# Autodesk Inventor assembly: Tamale - V1p5 - keepouts
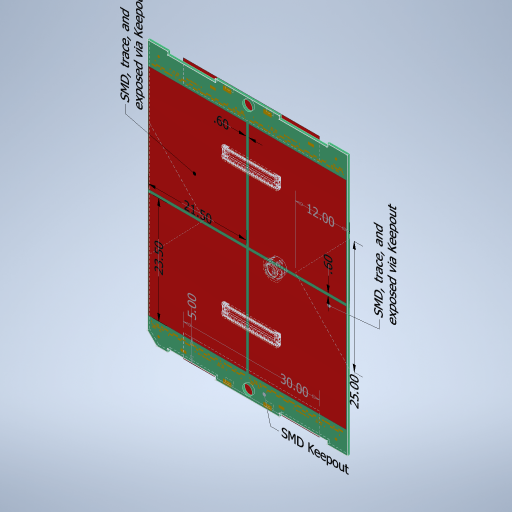
[picture p0: Inventor's stored thumbnail of the model, 512x512]
Saved by Autodesk Inventor 2023 (Build 270158000, 158)
## iProperties
Created: 2023-03-02
Part Number: Tamale - V1p5 - keepouts
Document SubType Name: Assembly
Designer: Caleb
Author: Caleb
## Documents named in this file (5)
- C:\Users\Caleb\Desktop\nebraska-silicon-lab\Hardware\ETL\modules\tamale v1.5\Tamale - V1p5 - keepouts.iam
- C:\Users\Caleb\Desktop\nebraska-silicon-lab\Hardware\ETL\modules\tamale v1.5\etl_module_pcb_mockup_v3p3p1.ipt
- C:\Users\Caleb\Desktop\nebraska-silicon-lab\Hardware\ETL\modules\tamale v1.5\keepout - bottom.ipt
- C:\Users\Caleb\Desktop\nebraska-silicon-lab\Hardware\ETL\modules\tamale v1.5\keepout - top A.ipt
- C:\Users\Caleb\Desktop\nebraska-silicon-lab\Hardware\ETL\modules\tamale v1.5\keepout - top B.ipt
## Components (6 placed, 4 different names)
1. etl_module_pcb_mockup_v3p3p1:1 — Mate:1, Angle:1, Flush:1, Flush:2, Mate:2, Flush:3, Mate:3, Flush:5, Mate:4, Mate:5, Flush:6, Flush:7, Mate:6, Mate:7
2. keepout - bottom:1 — Mate:1, Angle:1, Flush:1, Flush:2
3. keepout - top A:1 — Mate:2, Flush:3, Flush:4
4. keepout - top A:2 — Mate:3, Flush:4, Flush:5
5. keepout - top B:1 — Mate:4, Flush:6, Mate:6
6. keepout - top B:2 — Mate:5, Flush:7, Mate:7
## Relationships (15: Mate 7, Flush 7, Angle 1)
- Mate:1: etl_module_pcb_mockup_v3p3p1:1 ↔ keepout - bottom:1
- Angle:1 (0 deg): etl_module_pcb_mockup_v3p3p1:1 ↔ keepout - bottom:1
- Flush:1 (0.25 mm): etl_module_pcb_mockup_v3p3p1:1 ↔ keepout - bottom:1
- Flush:2 (4.95 mm): etl_module_pcb_mockup_v3p3p1:1 ↔ keepout - bottom:1
- Mate:2: etl_module_pcb_mockup_v3p3p1:1 ↔ keepout - top A:1
- Flush:3: etl_module_pcb_mockup_v3p3p1:1 ↔ keepout - top A:1
- Mate:3: etl_module_pcb_mockup_v3p3p1:1 ↔ keepout - top A:2
- Flush:4: keepout - top A:1 ↔ keepout - top A:2
- Flush:5: etl_module_pcb_mockup_v3p3p1:1 ↔ keepout - top A:2
- Mate:4: etl_module_pcb_mockup_v3p3p1:1 ↔ keepout - top B:1
- Mate:5: etl_module_pcb_mockup_v3p3p1:1 ↔ keepout - top B:2
- Flush:6: etl_module_pcb_mockup_v3p3p1:1 ↔ keepout - top B:1
- Flush:7: etl_module_pcb_mockup_v3p3p1:1 ↔ keepout - top B:2
- Mate:6 (-16.25 mm): etl_module_pcb_mockup_v3p3p1:1 ↔ keepout - top B:1
- Mate:7 (-16.25 mm): etl_module_pcb_mockup_v3p3p1:1 ↔ keepout - top B:2
